# Autodesk Inventor assembly: assy2
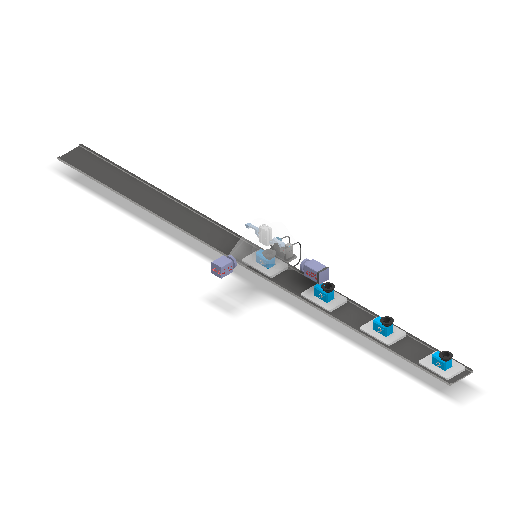
[picture p0: Inventor's stored thumbnail of the model, 512x512]
Saved by Autodesk Inventor 2025 (Build 290162000, 162)
## iProperties
Created: 2024-09-26
Part Number: assy2
Document SubType Name: Assembly
Designer: DMIADX
Author: DMIADX
## Documents named in this file (15)
- C:\Users\DMIADX\Documents\Inventor\chuck\assy2.iam
- C:\Users\DMIADX\Documents\Inventor\chuck\chuck.ipt
- C:\Users\DMIADX\Documents\Inventor\chuck\chuck_MIR.ipt
- C:\Users\DMIADX\Documents\Inventor\Content Center Files\R2025\en-US\ISO 4762(2)\ISO 4762 - M3 x 12ISO.ipt
- C:\Users\DMIADX\Documents\Inventor\chuck\pallet.ipt
- C:\Users\DMIADX\Documents\Inventor\chuck\part.ipt
- C:\Users\DMIADX\Documents\Inventor\chuck\CAMERA TERMINAL.ipt
- C:\Users\DMIADX\Documents\Inventor\chuck\CAMERA.ipt
- C:\Users\DMIADX\Documents\Inventor\chuck\flash.ipt
- C:\Users\DMIADX\Documents\Inventor\chuck\jalur.ipt
- C:\Users\DMIADX\Documents\Inventor\chuck\holder sensor.ipt
- C:\Users\DMIADX\Documents\Inventor\chuck\cover.ipt
- C:\Users\DMIADX\Documents\Inventor\chuck\sensor.ipt
- C:\Users\DMIADX\Documents\Inventor\chuck\MHZL2-20D\MHZL2-20D_LENGAN.ipt
- C:\Users\DMIADX\Documents\Inventor\chuck\CHUCKLENGAN.ipt
## Components (26 placed, 14 different names)
1. chuck:1 — Insert:1, Insert:2, Insert:11, Insert:12, Angle:2
2. chuck_MIR:1 — Insert:3, Insert:4, Insert:9, Insert:10, Angle:1
3. ISO 4762 M3 x 12:1 — Insert:1
4. ISO 4762 M3 x 12:2 — Insert:2
5. ISO 4762 M3 x 12:3 — Insert:4
6. ISO 4762 M3 x 12:4 — Insert:3
7. pallet:1 — Flush:7, geser palet, Mate:10, Mate:29
8. part:1 — part naik, Mate:43, Mate:44
9. pallet:2 — Mate:12, Flush:12, Flush:14, Mate:24
10. part:2 — Mate:13, Mate:45, Mate:46
11. CAMERA TERMINAL:1 — Flush:16, Mate:16, Flush:17, Insert:6
12. CAMERA:1 — Flush:15, Mate:14, Mate:15, Insert:5
13. flash:1 — Insert:5
14. flash:2 — Insert:6
15. jalur:1 — Mate:17, Mate:18, Flush:18, Mate:19, Mate:23, Mate:28, Mate:30, Mate:38, Flush:26
16. pallet:3 — Mate:19, Mate:22, Mate:23, Mate:24, Mate:48
17. part:3 — Mate:22, Mate:47, Mate:48
18. pallet:4 — Mate:28, Mate:29, Mate:30, Mate:41, Mate:42
19. part:4 — Mate:41, Mate:42
20. cover:1 — Mate:35, Mate:36, Mate:37, Flush:30
21. sensor:1 — Mate:39, Flush:28, Flush:29, Flush:31
22. sensor:2 — Mate:35, Mate:36, Mate:37, Mate:40, Flush:31
23. holder sensor:2 — Mate:38, Flush:26, Flush:27, Mate:39, Flush:28, Flush:29, Mate:40, Flush:30
24. MHZL2-20D_LENGAN:1 — Flush:32, Flush:33, Insert:7, Insert:8, Angle:1, Angle:2, Mate:49
25. CHUCKLENGAN:1 — Insert:7, Insert:11, Insert:12
26. CHUCKLENGAN:2 — Insert:8, Insert:9, Insert:10
## Relationships (62: Mate 32, Flush 16, Insert 12, Angle 2)
- Insert:1: chuck:1 ↔ ISO 4762 M3 x 12:1
- Insert:2: chuck:1 ↔ ISO 4762 M3 x 12:2
- Insert:3: chuck_MIR:1 ↔ ISO 4762 M3 x 12:4
- Insert:4: chuck_MIR:1 ↔ ISO 4762 M3 x 12:3
- Flush:7: pallet:1
- geser palet [Flush] (300 mm): pallet:1
- Mate:10: pallet:1
- part naik [Mate] (-8 mm): part:1
- Mate:43: part:1
- Mate:12: pallet:2
- Mate:13 (-8 mm): part:2
- Flush:12: pallet:2
- Flush:14 (600 mm): pallet:2
- Flush:15: CAMERA:1
- Mate:14 (-100 mm): CAMERA:1
- Mate:15 (250 mm): CAMERA:1
- Flush:16: CAMERA TERMINAL:1
- Mate:16 (-100 mm): CAMERA TERMINAL:1
- Flush:17 (300 mm): CAMERA TERMINAL:1
- Insert:5: CAMERA:1 ↔ flash:1
- Insert:6: CAMERA TERMINAL:1 ↔ flash:2
- Mate:17: jalur:1
- Mate:18: jalur:1
- Flush:18: jalur:1
- Mate:19: jalur:1 ↔ pallet:3
- Mate:22: pallet:3 ↔ part:3
- Mate:23: jalur:1 ↔ pallet:3
- Mate:24 (150 mm): pallet:2 ↔ pallet:3
- [Mate]: pallet:4 ↔ part:4
- Mate:28: jalur:1 ↔ pallet:4
- Mate:29 (150 mm): pallet:1 ↔ pallet:4
- Mate:30: jalur:1 ↔ pallet:4
- Mate:35: cover:1 ↔ sensor:2
- Mate:36: cover:1 ↔ sensor:2
- Mate:37: cover:1 ↔ sensor:2
- Mate:38: jalur:1 ↔ holder sensor:2
- Flush:26 (5 mm): jalur:1 ↔ holder sensor:2
- Flush:27: holder sensor:2
- Mate:39: sensor:1 ↔ holder sensor:2
- Flush:28 (3 mm): sensor:1 ↔ holder sensor:2
- Flush:29: sensor:1 ↔ holder sensor:2
- Mate:40: sensor:2 ↔ holder sensor:2
- Flush:30 (2 mm): cover:1 ↔ holder sensor:2
- Flush:31: sensor:1 ↔ sensor:2
- Flush:32: MHZL2-20D_LENGAN:1
- Flush:33: MHZL2-20D_LENGAN:1
- Insert:7: MHZL2-20D_LENGAN:1 ↔ CHUCKLENGAN:1
- Insert:8: MHZL2-20D_LENGAN:1 ↔ CHUCKLENGAN:2
- Insert:9: chuck_MIR:1 ↔ CHUCKLENGAN:2
- Insert:10: chuck_MIR:1 ↔ CHUCKLENGAN:2
- Insert:11: chuck:1 ↔ CHUCKLENGAN:1
- Insert:12: chuck:1 ↔ CHUCKLENGAN:1
- Angle:1 (0 deg): chuck_MIR:1 ↔ MHZL2-20D_LENGAN:1
- Angle:2 (0 deg): chuck:1 ↔ MHZL2-20D_LENGAN:1
- Mate:41: pallet:4 ↔ part:4
- Mate:42: pallet:4 ↔ part:4
- Mate:44 (-300 mm): part:1
- Mate:45: part:2
- Mate:46 (-600 mm): part:2
- Mate:47: part:3
- Mate:48: pallet:3 ↔ part:3
- Mate:49 (-165 mm): MHZL2-20D_LENGAN:1
## Named parameters: d63_d58 = 0 mm
